# Autodesk Inventor assembly: PWTR-0141
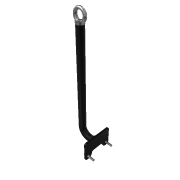
[picture p0: Inventor's stored thumbnail of the model, 180x180]
Saved by Autodesk Inventor 2021.1 (Build 251245000, 245)
## iProperties
Created: 2020-09-03
Part Number: PWTR-0141
Document SubType Name: Assembly
Designer: alid
Description: Lifting Arm Assembly
Author: alid
## Documents named in this file (4)
- C:\Vault Workspace\Design Data\Projects\PRJ0095\PWTR-CTO\PWTR-0141.iam
- C:\Vault Workspace\Design Data\Projects\PRJ0095\PWTR-CTO\PWTR-0140.ipt
- C:\Vault Workspace\Design Data\Projects\PRJ0095\PWTR-CTO\PWTR-0142.ipt
- C:\Vault Workspace\Design Data\Projects\PRJ0095\PWTR-CTO\PWTR-0143.ipt
## Components (4 placed, 3 different names)
1. Lifting Arm — Insert:1, Insert:2, Insert:3
2. PWTR-0142:1 — Insert:1
3. PWTR-0142:2 — Insert:2
4. Lifting Hook — Insert:3
## Relationships (3: Insert 3)
- Insert:1: Lifting Arm ↔ PWTR-0142:1
- Insert:2: Lifting Arm ↔ PWTR-0142:2
- Insert:3: Lifting Arm ↔ Lifting Hook
